# Autodesk Inventor assembly: uMule-elektronika
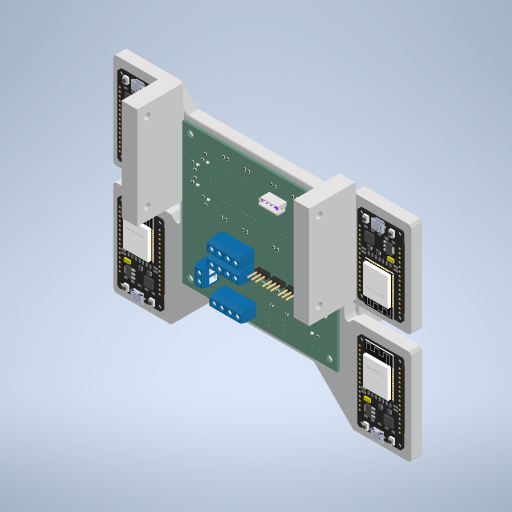
[picture p0: Inventor's stored thumbnail of the model, 512x512]
Saved by Autodesk Inventor 2024.2 (Build 282272000, 272)
## iProperties
Created: 2024-10-29
Part Number: uMule-elektronika
Document SubType Name: Assembly
Designer: owozn
Author: owozn
## Documents named in this file (4)
- C:\Users\owozn\Documents\Semestr 7\Inżynierka\Modele 3D\uMule-elektronika.iam
- C:\Users\owozn\Documents\Semestr 7\Inżynierka\Modele 3D\uMule-Main_board\uMule-Main_board.ipt
- C:\Users\owozn\Documents\Semestr 7\Inżynierka\Modele 3D\esp-10.snapshot.1\esp32\esp32.ipt
- C:\Users\owozn\Documents\Semestr 7\Inżynierka\Modele 3D\uMule-podstawa_elektronika.ipt
## Components (6 placed, 3 different names)
1. uMule-Main_board:1 — Równoległe:1, Równoległe:2, Równoległe:3, Równoległe:4, Zestawiające:7, Zestawiające:8, Zestawiające:9
2. esp32:1 — Równoległe:4, Zestawiające:6, Zestawiające:10
3. esp32:2 — Równoległe:3, Zestawiające:6, Równoległe:5, Zestawiające:12
4. esp32:3 — Równoległe:1, Zestawiające:5, Równoległe:5, Równoległe:6
5. esp32:4 — Równoległe:2, Zestawiające:5, Zestawiające:11, Równoległe:6
6. uMule-podstawa_elektronika:1 — Zestawiające:7, Zestawiające:8, Zestawiające:9, Zestawiające:10, Zestawiające:11, Zestawiające:12
## Relationships (14: Mate 8, Flush 6)
- Równoległe:1 [Flush]: uMule-Main_board:1 ↔ esp32:3
- Równoległe:2 [Flush]: uMule-Main_board:1 ↔ esp32:4
- Równoległe:3 [Flush]: uMule-Main_board:1 ↔ esp32:2
- Równoległe:4 [Flush]: uMule-Main_board:1 ↔ esp32:1
- Zestawiające:5 [Mate] (20 mm): esp32:3 ↔ esp32:4
- Zestawiające:6 [Mate] (20 mm): esp32:1 ↔ esp32:2
- Równoległe:5 [Flush]: esp32:2 ↔ esp32:3
- Zestawiające:7 [Mate]: uMule-Main_board:1 ↔ uMule-podstawa_elektronika:1
- Zestawiające:8 [Mate]: uMule-Main_board:1 ↔ uMule-podstawa_elektronika:1
- Zestawiające:9 [Mate]: uMule-Main_board:1 ↔ uMule-podstawa_elektronika:1
- Zestawiające:10 [Mate]: esp32:1 ↔ uMule-podstawa_elektronika:1
- Zestawiające:11 [Mate]: esp32:4 ↔ uMule-podstawa_elektronika:1
- Zestawiające:12 [Mate]: esp32:2 ↔ uMule-podstawa_elektronika:1
- Równoległe:6 [Flush]: esp32:3 ↔ esp32:4
